# Autodesk Inventor assembly: Cylinder
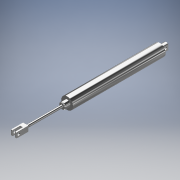
[picture p0: Inventor's stored thumbnail of the model, 180x180]
Saved by Autodesk Inventor 2017 SP1 (Build 210196100, 196)
## iProperties
Created: 2018-01-27
Part Number: Cylinder
Document SubType Name: Assembly
Designer: Ben
Author: Ben
## Documents named in this file (3)
- C:\Users\Ben\Desktop\Projects\2018 Robot\Cube Lift\Cylinder.iam
- C:\Users\Ben\Desktop\Projects\2018 Robot\Cube Lift\cylinder body.ipt
- C:\Users\Ben\Desktop\Projects\2018 Robot\Cube Lift\cylinder piston.ipt
## Components (2 placed, 2 different names)
1. cylinder body:1 — Mate:1
2. cylinder piston:1 — Mate:1
## Relationships (1: Mate 1)
- Mate:1: cylinder body:1 ↔ cylinder piston:1
